# Autodesk Inventor assembly: Assembly1
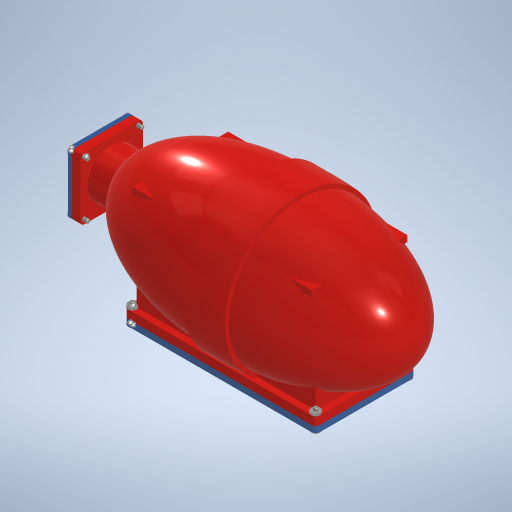
[picture p0: Inventor's stored thumbnail of the model, 512x512]
Saved by Autodesk Inventor 2023 (Build 270158000, 158)
## iProperties
Created: 2023-03-23
Part Number: Assembly1
Document SubType Name: Assembly
Designer: andre
Author: andre
## Documents named in this file (10)
- C:\Users\andre\OneDrive\Desktop\Diseño-del-submarino-ANDRES\Diseño del submarino\Assembly1.iam
- C:\Users\andre\OneDrive\Desktop\Prototipo 1\Prototipo 1\Caparazon_rosca_1.ipt
- C:\Users\andre\OneDrive\Desktop\Prototipo 1\Prototipo 1\Caparazon_rosca_2.ipt
- C:\Users\andre\OneDrive\Desktop\Prototipo 1\Prototipo 1\Capsula.ipt
- C:\Users\andre\OneDrive\Desktop\Prototipo 1\Prototipo 1\Tapa principal.ipt
- C:\Users\andre\OneDrive\Desktop\Prototipo 1\Prototipo 1\Tapa trasera.ipt
- C:\Users\andre\OneDrive\Documents\Inventor\Content Center Files\R2023\en-US\ANSI B18.6.3(28)\ANSI B18.6.3 - 1-64 UNC - 0.375(12).ipt
- C:\Users\andre\OneDrive\Documents\Inventor\Content Center Files\R2023\en-US\ASME B18.6.3\ASME B18.6.3 - 1-64.ipt
- C:\Users\andre\OneDrive\Documents\Inventor\Content Center Files\R2023\en-US\ANSI B18.6.3(28)\ANSI B18.6.3 - 1-64 UNC - 0.3125(12).ipt
- C:\Users\andre\OneDrive\Documents\Inventor\Content Center Files\R2023\en-US\ANSI B18.6.3(26)\ANSI B18.6.3 - 1-64 UNC - 0.3125(7).ipt
## Components (17 placed, 9 different names)
1. Caparazon_rosca_1:1 — Rotational:1, Mate:1, Mate:38, Mate:40, Mate:41, Mate:46, Mate:48, Mate:49
2. Caparazon_rosca_2:1 — Rotational:1, Rigid:1, Mate:2, Mate:3, Rigid:2, Mate:37, Mate:45
3. Capsula:1 — Rigid:1
4. Tapa principal:1 — Mate:1, Mate:2, Mate:3, Mate:34, Mate:35, Mate:36, Mate:39, Mate:42, Mate:43, Mate:44, Mate:47
5. Tapa trasera:1 — Rigid:2, Mate:10, Mate:11, Mate:16, Mate:17, Mate:18, Mate:19, Mate:20, Mate:21
6. Cross Recessed Truss Head Machine Screw - Type IA - Inch 1 - 64 - 5/16:1 — Mate:10, Mate:11
7. Cross Recessed Truss Head Machine Screw - Type IA - Inch 1 - 64 - 5/16:2 — Mate:16, Mate:17
8. Cross Recessed Pan Head Machine Screw - Type II - Inch 1 - 64 - 5/16:1 — Mate:18, Mate:19
9. Cross Recessed Truss Head Machine Screw - Type IA - Inch 1 - 64 - 5/16:3 — Mate:20, Mate:21
10. Cross Recessed Truss Head Machine Screw - Type IA - Inch No. 1 - 64 - 3/8:1 — Mate:34, Mate:35
11. Chamfered Bottom Hex Machine Screw Nuts 1-64:1 — Mate:36, Mate:37
12. Cross Recessed Truss Head Machine Screw - Type IA - Inch No. 1 - 64 - 3/8:2 — Mate:38, Mate:39
13. Chamfered Bottom Hex Machine Screw Nuts 1-64:2 — Mate:40, Mate:41
14. Cross Recessed Truss Head Machine Screw - Type IA - Inch No. 1 - 64 - 3/8:3 — Mate:42, Mate:43
15. Chamfered Bottom Hex Machine Screw Nuts 1-64:3 — Mate:44, Mate:45
16. Cross Recessed Truss Head Machine Screw - Type IA - Inch No. 1 - 64 - 3/8:4 — Mate:46, Mate:47
17. Chamfered Bottom Hex Machine Screw Nuts 1-64:4 — Mate:48, Mate:49
## Relationships (30: Mate 27, WeldJoint 2, RevoluteJoint 1)
- Rotational:1 [RevoluteJoint]: Caparazon_rosca_1:1 ↔ Caparazon_rosca_2:1
- Rigid:1 [WeldJoint]: Caparazon_rosca_2:1 ↔ Capsula:1
- Mate:1: Caparazon_rosca_1:1 ↔ Tapa principal:1
- Mate:2: Caparazon_rosca_2:1 ↔ Tapa principal:1
- Mate:3: Caparazon_rosca_2:1 ↔ Tapa principal:1
- Rigid:2 [WeldJoint]: Caparazon_rosca_2:1 ↔ Tapa trasera:1
- Mate:10: Tapa trasera:1 ↔ Cross Recessed Truss Head Machine Screw - Type IA - Inch 1 - 64 - 5/16:1
- Mate:11: Tapa trasera:1 ↔ Cross Recessed Truss Head Machine Screw - Type IA - Inch 1 - 64 - 5/16:1
- Mate:16: Tapa trasera:1 ↔ Cross Recessed Truss Head Machine Screw - Type IA - Inch 1 - 64 - 5/16:2
- Mate:17: Tapa trasera:1 ↔ Cross Recessed Truss Head Machine Screw - Type IA - Inch 1 - 64 - 5/16:2
- Mate:18: Tapa trasera:1 ↔ Cross Recessed Pan Head Machine Screw - Type II - Inch 1 - 64 - 5/16:1
- Mate:19: Tapa trasera:1 ↔ Cross Recessed Pan Head Machine Screw - Type II - Inch 1 - 64 - 5/16:1
- Mate:20: Tapa trasera:1 ↔ Cross Recessed Truss Head Machine Screw - Type IA - Inch 1 - 64 - 5/16:3
- Mate:21: Tapa trasera:1 ↔ Cross Recessed Truss Head Machine Screw - Type IA - Inch 1 - 64 - 5/16:3
- Mate:34: Tapa principal:1 ↔ Cross Recessed Truss Head Machine Screw - Type IA - Inch No. 1 - 64 - 3/8:1
- Mate:35: Tapa principal:1 ↔ Cross Recessed Truss Head Machine Screw - Type IA - Inch No. 1 - 64 - 3/8:1
- Mate:36: Tapa principal:1 ↔ Chamfered Bottom Hex Machine Screw Nuts 1-64:1
- Mate:37: Caparazon_rosca_2:1 ↔ Chamfered Bottom Hex Machine Screw Nuts 1-64:1
- Mate:38: Caparazon_rosca_1:1 ↔ Cross Recessed Truss Head Machine Screw - Type IA - Inch No. 1 - 64 - 3/8:2
- Mate:39: Tapa principal:1 ↔ Cross Recessed Truss Head Machine Screw - Type IA - Inch No. 1 - 64 - 3/8:2
- Mate:40: Caparazon_rosca_1:1 ↔ Chamfered Bottom Hex Machine Screw Nuts 1-64:2
- Mate:41: Caparazon_rosca_1:1 ↔ Chamfered Bottom Hex Machine Screw Nuts 1-64:2
- Mate:42: Tapa principal:1 ↔ Cross Recessed Truss Head Machine Screw - Type IA - Inch No. 1 - 64 - 3/8:3
- Mate:43: Tapa principal:1 ↔ Cross Recessed Truss Head Machine Screw - Type IA - Inch No. 1 - 64 - 3/8:3
- Mate:44: Tapa principal:1 ↔ Chamfered Bottom Hex Machine Screw Nuts 1-64:3
- Mate:45: Caparazon_rosca_2:1 ↔ Chamfered Bottom Hex Machine Screw Nuts 1-64:3
- Mate:46: Caparazon_rosca_1:1 ↔ Cross Recessed Truss Head Machine Screw - Type IA - Inch No. 1 - 64 - 3/8:4
- Mate:47: Tapa principal:1 ↔ Cross Recessed Truss Head Machine Screw - Type IA - Inch No. 1 - 64 - 3/8:4
- Mate:48: Caparazon_rosca_1:1 ↔ Chamfered Bottom Hex Machine Screw Nuts 1-64:4
- Mate:49: Caparazon_rosca_1:1 ↔ Chamfered Bottom Hex Machine Screw Nuts 1-64:4
